# Autodesk Inventor assembly: prostkatna waska wysoka
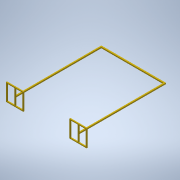
[picture p0: Inventor's stored thumbnail of the model, 180x180]
Saved by Autodesk Inventor 2021 (Build 250183000, 183)
## iProperties
Created: 2024-04-18
Part Number: prostkatna waska wysoka
Document SubType Name: Assembly
Designer: Michal
Author: Michal
## Documents named in this file (7)
- C:\Users\Michal\Documents\GitHub\PNW_PhotoBoothFrame_3D\prostkatna waska wysoka.iam
- C:\Users\Michal\Documents\GitHub\PNW_PhotoBoothFrame_3D\M8x15.ipt
- C:\Users\Michal\Documents\GitHub\PNW_PhotoBoothFrame_3D\Gora L1500.ipt
- C:\Users\Michal\Documents\GitHub\PNW_PhotoBoothFrame_3D\Noga L L2000.ipt
- C:\Users\Michal\Documents\GitHub\PNW_PhotoBoothFrame_3D\Noga P L2000.ipt
- C:\Users\Michal\Documents\GitHub\PNW_PhotoBoothFrame_3D\Naroznik.iam
- C:\Users\Michal\Documents\GitHub\PNW_PhotoBoothFrame_3D\Stopa v1.iam
## Components (19 placed, 6 different names)
1. Stopa v1:1 [sub-assembly] — Flush:1, Flush:2, Mate:1, Flush:3, Mate:2, Mate:3, Mate:5
2. Stopa v1:2 [sub-assembly] — Flush:1, Flush:2, Mate:10, Flush:4, Flush:5, Mate:11, Mate:18, Mate:20
3. Naroznik:1 [sub-assembly] — Mate:12, Mate:13, Mate:14, Mate:15, Mate:22, Mate:24, Mate:26, Mate:28
4. Naroznik:2 [sub-assembly] — Mate:7, Mate:8, Mate:9, Mate:17, Mate:30, Mate:32, Mate:34, Mate:36
5. Noga L L2000:1 — Mate:1, Flush:3, Mate:2, Mate:4, Mate:6, Mate:7, Mate:8, Mate:9, Mate:31, Mate:33
6. M8x15:1 — Mate:3, Mate:4
7. M8x15:2 — Mate:5, Mate:6
8. Noga P L2000:1 — Mate:10, Flush:4, Flush:5, Mate:11, Mate:12, Mate:13, Mate:14, Flush:6, Mate:19, Mate:21, Mate:23, Mate:25
9. Gora L1500:1 — Flush:6, Mate:15, Mate:17, Mate:27, Mate:29, Mate:35, Mate:37, Mate:38, Flush:7, Mate:39
10. M8x15:3 — Mate:18, Mate:19
11. M8x15:4 — Mate:20, Mate:21
12. M8x15:5 — Mate:22, Mate:23
13. M8x15:6 — Mate:24, Mate:25
14. M8x15:7 — Mate:26, Mate:27
15. M8x15:8 — Mate:28, Mate:29
16. M8x15:9 — Mate:30, Mate:31
17. M8x15:10 — Mate:32, Mate:33
18. M8x15:11 — Mate:34, Mate:35
19. M8x15:12 — Mate:36, Mate:37
## Relationships (45: Mate 38, Flush 7)
- Flush:1: Stopa v1:1 ↔ Stopa v1:2
- Flush:2: Stopa v1:1 ↔ Stopa v1:2
- Mate:1: Stopa v1:1 ↔ Noga L L2000:1
- Flush:3: Stopa v1:1 ↔ Noga L L2000:1
- Mate:2: Stopa v1:1 ↔ Noga L L2000:1
- Mate:3: Stopa v1:1 ↔ M8x15:1
- Mate:4: Noga L L2000:1 ↔ M8x15:1
- Mate:5: Stopa v1:1 ↔ M8x15:2
- Mate:6: Noga L L2000:1 ↔ M8x15:2
- Mate:7: Naroznik:2 ↔ Noga L L2000:1
- Mate:8: Naroznik:2 ↔ Noga L L2000:1
- Mate:9: Naroznik:2 ↔ Noga L L2000:1
- Mate:10: Stopa v1:2 ↔ Noga P L2000:1
- Flush:4: Stopa v1:2 ↔ Noga P L2000:1
- Flush:5: Stopa v1:2 ↔ Noga P L2000:1
- Mate:11: Stopa v1:2 ↔ Noga P L2000:1
- Mate:12: Naroznik:1 ↔ Noga P L2000:1
- Mate:13: Naroznik:1 ↔ Noga P L2000:1
- Mate:14: Naroznik:1 ↔ Noga P L2000:1
- Flush:6: Noga P L2000:1 ↔ Gora L1500:1
- Mate:15: Naroznik:1 ↔ Gora L1500:1
- Mate:17: Naroznik:2 ↔ Gora L1500:1
- Mate:18: Stopa v1:2 ↔ M8x15:3
- Mate:19: Noga P L2000:1 ↔ M8x15:3
- Mate:20: Stopa v1:2 ↔ M8x15:4
- Mate:21: Noga P L2000:1 ↔ M8x15:4
- Mate:22: Naroznik:1 ↔ M8x15:5
- Mate:23: Noga P L2000:1 ↔ M8x15:5
- Mate:24: Naroznik:1 ↔ M8x15:6
- Mate:25: Noga P L2000:1 ↔ M8x15:6
- Mate:26: Naroznik:1 ↔ M8x15:7
- Mate:27: Gora L1500:1 ↔ M8x15:7
- Mate:28: Naroznik:1 ↔ M8x15:8
- Mate:29: Gora L1500:1 ↔ M8x15:8
- Mate:30: Naroznik:2 ↔ M8x15:9
- Mate:31: Noga L L2000:1 ↔ M8x15:9
- Mate:32: Naroznik:2 ↔ M8x15:10
- Mate:33: Noga L L2000:1 ↔ M8x15:10
- Mate:34: Naroznik:2 ↔ M8x15:11
- Mate:35: Gora L1500:1 ↔ M8x15:11
- Mate:36: Naroznik:2 ↔ M8x15:12
- Mate:37: Gora L1500:1 ↔ M8x15:12
- Mate:38: Gora L1500:1
- Flush:7: Gora L1500:1
- Mate:39: Gora L1500:1
